# Autodesk Inventor assembly: Lifting Platform Assembly
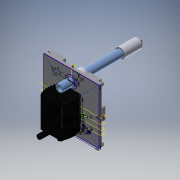
[picture p0: Inventor's stored thumbnail of the model, 180x180]
Saved by Autodesk Inventor 2016 (Build 200138000, 138)
## iProperties
Created: 2016-05-06
Part Number: Lifting Platform Assembly
Document SubType Name: Assembly
Designer: Kenneth Daniel
Author: Kenneth Daniel
## Documents named in this file (4)
- C:\Users\Kenneth Daniel\Documents\Enes 100A\Final Prints and Versions\Lifting Platform Assembly.iam
- C:\Users\Kenneth Daniel\Documents\Enes 100A\Final Prints and Versions\Complete Lifting Chassis with Balance and Variability.ipt
- C:\Users\Kenneth Daniel\Documents\Enes 100A\Final Prints and Versions\To Much Work, Motor.ipt
- C:\Users\Kenneth Daniel\Documents\Enes 100A\Final Prints and Versions\PH Monitor.ipt
## Components (3 placed, 3 different names)
1. Complete Lifting Chassis with Balance and Variability:1 — Mate:1, Mate:2, Mate:3
2. To Much Work, Motor:1 — Mate:3
3. PH Monitor:1 — Mate:1, Mate:2
## Relationships (3: Mate 3)
- Mate:1: Complete Lifting Chassis with Balance and Variability:1 ↔ PH Monitor:1
- Mate:2: Complete Lifting Chassis with Balance and Variability:1 ↔ PH Monitor:1
- Mate:3: Complete Lifting Chassis with Balance and Variability:1 ↔ To Much Work, Motor:1
